# Autodesk Inventor assembly: withBase
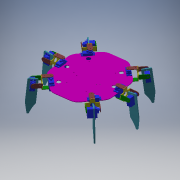
[picture p0: Inventor's stored thumbnail of the model, 180x180]
Saved by Autodesk Inventor 2019.1 (Build 231200000, 200)
## iProperties
Created: 2018-12-04
Part Number: withBase
Document SubType Name: Assembly
Designer: kfortuna
Author: kfortuna
## Documents named in this file (3)
- C:\Users\kfortuna\Desktop\withBase.iam
- C:\Users\kfortuna\Desktop\Base.ipt
- C:\Users\kfortuna\Desktop\legAssembly.iam
## Components (7 placed, 2 different names)
1. Base:1 — Mate:1, Flush:1, Mate:2, Mate:3, Mate:4, Flush:2, Mate:6, Mate:7, Flush:3, Mate:9, Mate:10, Flush:4, Mate:11, Flush:5, Mate:12, Mate:13, Mate:14, Mate:15
2. legAssembly:1 [sub-assembly] — Mate:13, Mate:14, Mate:15
3. legAssembly:2 [sub-assembly] — Mate:11, Flush:5, Mate:12
4. legAssembly:3 [sub-assembly] — Mate:9, Mate:10, Flush:4
5. legAssembly:4 [sub-assembly] — Mate:6, Mate:7, Flush:3
6. legAssembly:5 [sub-assembly] — Mate:3, Mate:4, Flush:2
7. legAssembly:6 [sub-assembly] — Mate:1, Flush:1, Mate:2
## Relationships (18: Mate 13, Flush 5)
- Mate:1: Base:1 ↔ legAssembly:6
- Flush:1: Base:1 ↔ legAssembly:6
- Mate:2: Base:1 ↔ legAssembly:6
- Mate:3: Base:1 ↔ legAssembly:5
- Mate:4: Base:1 ↔ legAssembly:5
- Flush:2: Base:1 ↔ legAssembly:5
- Mate:6: Base:1 ↔ legAssembly:4
- Mate:7: Base:1 ↔ legAssembly:4
- Flush:3: Base:1 ↔ legAssembly:4
- Mate:9: Base:1 ↔ legAssembly:3
- Mate:10: Base:1 ↔ legAssembly:3
- Flush:4: Base:1 ↔ legAssembly:3
- Mate:11: Base:1 ↔ legAssembly:2
- Flush:5: Base:1 ↔ legAssembly:2
- Mate:12: Base:1 ↔ legAssembly:2
- Mate:13: Base:1 ↔ legAssembly:1
- Mate:14: Base:1 ↔ legAssembly:1
- Mate:15: Base:1 ↔ legAssembly:1
